# Autodesk Inventor assembly: Claw2017-18
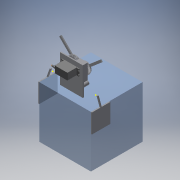
[picture p0: Inventor's stored thumbnail of the model, 180x180]
Saved by Autodesk Inventor 2017 (Build 210142000, 142)
## iProperties
Created: 2017-09-28
Part Number: Claw2017-18
Document SubType Name: Assembly
Designer: User
Author: User
## Documents named in this file (8)
- C:\Robotics\CAD\2017-18_CAD\Claw2017-18.iam
- C:\Robotics\CAD\2017-18_CAD\ClawPaddle.ipt
- C:\Robotics\CAD\2017-18_CAD\ClawServoHolder.ipt
- C:\Robotics\CAD\COTSParts\Tetrix\Tetrix servo 180.ipt
- C:\Robotics\CAD\2017-18_CAD\Glyph6x6x6.ipt
- C:\Robotics\CAD\COTSParts\Tetrix\Tetrix Gear 40T.ipt
- C:\Robotics\CAD\COTSParts\Vex\91259A574_ALLOY STEEL SHOULDER SCREW.ipt
- C:\Robotics\CAD\2017-18_CAD\ClawLinkage.ipt
## Components (10 placed, 7 different names)
1. ClawPaddle:1 — Flush:1, Flush:2, Mate:4, Flush:3, Flush:4
2. ClawPaddle:2 — Flush:1, Flush:2, Mate:3
3. ClawServoHolder:1 — Mate:5, Mate:6, Mate:7, Mate:11, Mate:12, Flush:6, Mate:25
4. Tetrix servo 180:1 — Mate:5, Mate:6, Mate:7, Mate:9, Mate:10
5. Glyph6x6x6:1 — Mate:3, Mate:4, Flush:3, Flush:4, Flush:6, Mate:25
6. Tetrix Gear 40T:1 — Mate:9, Mate:10, Flush:5, Mate:19, Mate:20, Mate:21
7. Tetrix Gear 40T:2 — Mate:11, Mate:12, Flush:5, Mate:13, Mate:14, Mate:22, Mate:23, Mate:24
8. 91259A574_ALLOY STEEL SHOULDER SCREW:1 — Mate:13, Mate:14
9. ClawLinkage:1 — Mate:19, Mate:20, Mate:21
10. ClawLinkage:2 — Mate:22, Mate:23, Mate:24
## Relationships (24: Mate 18, Flush 6)
- Flush:1: ClawPaddle:1 ↔ ClawPaddle:2
- Flush:2: ClawPaddle:1 ↔ ClawPaddle:2
- Mate:3: ClawPaddle:2 ↔ Glyph6x6x6:1
- Mate:4: ClawPaddle:1 ↔ Glyph6x6x6:1
- Flush:3: ClawPaddle:1 ↔ Glyph6x6x6:1
- Flush:4: ClawPaddle:1 ↔ Glyph6x6x6:1
- Mate:5: ClawServoHolder:1 ↔ Tetrix servo 180:1
- Mate:6: ClawServoHolder:1 ↔ Tetrix servo 180:1
- Mate:7: ClawServoHolder:1 ↔ Tetrix servo 180:1
- Mate:9: Tetrix servo 180:1 ↔ Tetrix Gear 40T:1
- Mate:10: Tetrix servo 180:1 ↔ Tetrix Gear 40T:1
- Mate:11: ClawServoHolder:1 ↔ Tetrix Gear 40T:2
- Mate:12: ClawServoHolder:1 ↔ Tetrix Gear 40T:2
- Flush:5: Tetrix Gear 40T:1 ↔ Tetrix Gear 40T:2
- Flush:6 (47.6123 mm): ClawServoHolder:1 ↔ Glyph6x6x6:1
- Mate:13: Tetrix Gear 40T:2 ↔ 91259A574_ALLOY STEEL SHOULDER SCREW:1
- Mate:14: Tetrix Gear 40T:2 ↔ 91259A574_ALLOY STEEL SHOULDER SCREW:1
- Mate:19: Tetrix Gear 40T:1 ↔ ClawLinkage:1
- Mate:20: Tetrix Gear 40T:1 ↔ ClawLinkage:1
- Mate:21: Tetrix Gear 40T:1 ↔ ClawLinkage:1
- Mate:22: Tetrix Gear 40T:2 ↔ ClawLinkage:2
- Mate:23: Tetrix Gear 40T:2 ↔ ClawLinkage:2
- Mate:24: Tetrix Gear 40T:2 ↔ ClawLinkage:2
- Mate:25: ClawServoHolder:1 ↔ Glyph6x6x6:1
